# Autodesk Inventor assembly: spool
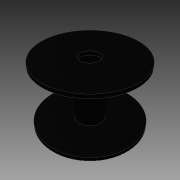
[picture p0: Inventor's stored thumbnail of the model, 180x180]
Saved by Autodesk Inventor 2014 (Build 180170000, 170)
## iProperties
Created: 2013-12-11
Part Number: spool
Document SubType Name: Assembly
Designer: buben
Author: buben
## Documents named in this file (3)
- C:\Users\buben\Documents\GitHub\bacon\inventor files\utils\spool.iam
- C:\Users\buben\Documents\GitHub\bacon\inventor files\utils\spool_side.ipt
- C:\Users\buben\Documents\GitHub\bacon\inventor files\utils\spool_core.ipt
## Components (3 placed, 2 different names)
1. spool_side:1 — Mate:1, Mate:2
2. spool_side:2 — Mate:3, Mate:4
3. spool_core:1 — Mate:1, Mate:2, Mate:3, Mate:4
## Relationships (4: Mate 4)
- Mate:1: spool_side:1 ↔ spool_core:1
- Mate:2: spool_side:1 ↔ spool_core:1
- Mate:3: spool_side:2 ↔ spool_core:1
- Mate:4: spool_side:2 ↔ spool_core:1
